# Autodesk Inventor assembly: Y Axis
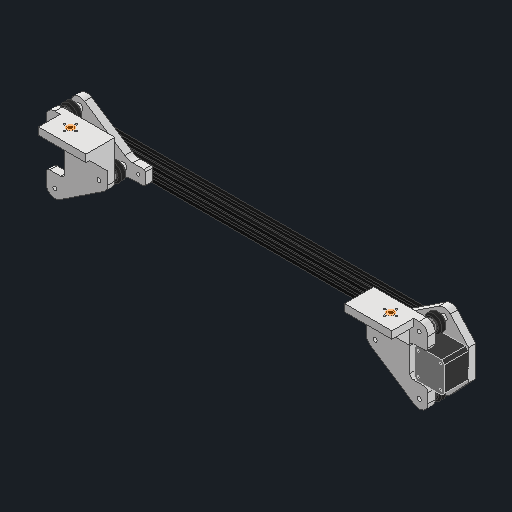
[picture p0: Inventor's stored thumbnail of the model, 512x512]
Saved by Autodesk Inventor 2025.1 (Build 291241000, 241)
## iProperties
Created: 2025-02-05
Part Number: Y Axis
Document SubType Name: Assembly
Designer: jerem
Author: jerem
## Documents named in this file (10)
- C:\Users\jerem\Documents\GitHub\Perovskite-Automated-Synthesis-System\CAD\Gantry\Y Axis.iam
- C:\Users\jerem\Documents\GitHub\Perovskite-Automated-Synthesis-System\CAD\Non 3D Printed Parts\Extrusion\V Extrustion 20x500mm.ipt
- C:\Users\jerem\Documents\GitHub\Perovskite-Automated-Synthesis-System\CAD\Gantry\y axis motor holder.ipt
- C:\Users\jerem\Documents\GitHub\Perovskite-Automated-Synthesis-System\CAD\Gantry\y axis something back.ipt
- C:\Users\jerem\Documents\GitHub\Perovskite-Automated-Synthesis-System\CAD\Gantry\y axis something.ipt
- C:\Users\jerem\Documents\GitHub\Perovskite-Automated-Synthesis-System\CAD\Non 3D Printed Parts\Motors and Servos\NEMA17 Stepper Motor.ipt
- C:\Users\jerem\Documents\GitHub\Perovskite-Automated-Synthesis-System\CAD\Non 3D Printed Parts\Printer Wheel.ipt
- C:\Users\jerem\Documents\GitHub\Perovskite-Automated-Synthesis-System\CAD\Gantry\y axis something_MIR.ipt
- C:\Users\jerem\Documents\GitHub\Perovskite-Automated-Synthesis-System\CAD\Non 3D Printed Parts\Leadscrew.ipt
- C:\Users\jerem\Documents\GitHub\Perovskite-Automated-Synthesis-System\CAD\Gantry\Y Axis Spacer.ipt
## Components (26 placed, 9 different names)
1. V Extrustion 20x500mm:1 — Mate:14, Mate:24, Mate:25, Mate:26, Flush:1
2. y axis motor holder:1 — Mate:1, Mate:2, Mate:4, Mate:5, Mate:7, Mate:8, Mate:9, Mate:13, Mate:14, Mate:25, Mate:36, Mate:37, Mate:38, Mate:49, Mate:50, Flush:1
3. y axis something back:1 — Mate:21, Mate:22, Mate:24, Mate:26, Mate:39, Mate:40, Mate:41, Mate:58, Mate:59, Mate:60
4. y axis something:1 — Mate:4, Mate:5, Mate:30, Mate:31, Mate:32, Mate:33, Mate:34, Mate:35, Mate:46, Mate:47, Mate:48
5. NEMA17 Stepper Motor:1 — Mate:1, Mate:2, Mate:13
6. Printer Wheel:1 — Mate:7, Mate:54
7. Printer Wheel:2 — Mate:8, Mate:53
8. Printer Wheel:3 — Mate:9, Mate:45, Mate:51, Mate:52
9. y axis something_MIR:1 — Mate:16, Mate:17, Mate:18, Mate:21, Mate:22, Mate:27, Mate:28, Mate:29, Mate:42, Mate:43, Mate:44, Mate:55, Mate:56, Mate:57
10. Printer Wheel:4 — Mate:18, Mate:63, Mate:64
11. Printer Wheel:5 — Mate:17, Mate:62
12. Printer Wheel:6 — Mate:16, Mate:61
13. Leadscrew:1 — Mate:27, Mate:28, Mate:29
14. Leadscrew:2 — Mate:30, Mate:31, Mate:32
15. Y Axis Spacer:1 — Mate:37, Mate:49, Mate:54
16. Y Axis Spacer:2 — Mate:38, Mate:50, Mate:53
17. Y Axis Spacer:3 — Mate:36, Mate:45, Mate:51
18. Y Axis Spacer:4 — Mate:41, Mate:59, Mate:64
19. Y Axis Spacer:5 — Mate:43, Mate:55, Mate:62
20. Y Axis Spacer:6 — Mate:42, Mate:56, Mate:61
21. Y Axis Spacer:7 — Mate:40, Mate:58
22. Y Axis Spacer:8 — Mate:39, Mate:60
23. Y Axis Spacer:9 — Mate:44, Mate:57, Mate:63
24. Y Axis Spacer:10 — Mate:34, Mate:47
25. Y Axis Spacer:11 — Mate:35, Mate:46, Mate:52
26. Y Axis Spacer:12 — Mate:33, Mate:48
## Relationships (56: Mate 55, Flush 1)
- Mate:1: y axis motor holder:1 ↔ NEMA17 Stepper Motor:1
- Mate:2: y axis motor holder:1 ↔ NEMA17 Stepper Motor:1
- Mate:4: y axis motor holder:1 ↔ y axis something:1
- Mate:5: y axis motor holder:1 ↔ y axis something:1
- Mate:7: y axis motor holder:1 ↔ Printer Wheel:1
- Mate:8: y axis motor holder:1 ↔ Printer Wheel:2
- Mate:9: y axis motor holder:1 ↔ Printer Wheel:3
- Mate:13: y axis motor holder:1 ↔ NEMA17 Stepper Motor:1
- Mate:14: V Extrustion 20x500mm:1 ↔ y axis motor holder:1
- Mate:16: y axis something_MIR:1 ↔ Printer Wheel:6
- Mate:17: y axis something_MIR:1 ↔ Printer Wheel:5
- Mate:18: y axis something_MIR:1 ↔ Printer Wheel:4
- Mate:21: y axis something back:1 ↔ y axis something_MIR:1
- Mate:22: y axis something back:1 ↔ y axis something_MIR:1
- Mate:24: V Extrustion 20x500mm:1 ↔ y axis something back:1
- Mate:25: V Extrustion 20x500mm:1 ↔ y axis motor holder:1
- Mate:26: V Extrustion 20x500mm:1 ↔ y axis something back:1
- Mate:27: y axis something_MIR:1 ↔ Leadscrew:1
- Mate:28: y axis something_MIR:1 ↔ Leadscrew:1
- Mate:29: y axis something_MIR:1 ↔ Leadscrew:1
- Mate:30: y axis something:1 ↔ Leadscrew:2
- Mate:31: y axis something:1 ↔ Leadscrew:2
- Mate:32: y axis something:1 ↔ Leadscrew:2
- Mate:33: y axis something:1 ↔ Y Axis Spacer:12
- Mate:34: y axis something:1 ↔ Y Axis Spacer:10
- Mate:35: y axis something:1 ↔ Y Axis Spacer:11
- Mate:36: y axis motor holder:1 ↔ Y Axis Spacer:3
- Mate:37: y axis motor holder:1 ↔ Y Axis Spacer:1
- Mate:38: y axis motor holder:1 ↔ Y Axis Spacer:2
- Mate:39: y axis something back:1 ↔ Y Axis Spacer:8
- Mate:40: y axis something back:1 ↔ Y Axis Spacer:7
- Mate:41: y axis something back:1 ↔ Y Axis Spacer:4
- Mate:42: y axis something_MIR:1 ↔ Y Axis Spacer:6
- Mate:43: y axis something_MIR:1 ↔ Y Axis Spacer:5
- Mate:44: y axis something_MIR:1 ↔ Y Axis Spacer:9
- Mate:45: Printer Wheel:3 ↔ Y Axis Spacer:3
- Mate:46: y axis something:1 ↔ Y Axis Spacer:11
- Mate:47: y axis something:1 ↔ Y Axis Spacer:10
- Mate:48: y axis something:1 ↔ Y Axis Spacer:12
- Mate:49: y axis motor holder:1 ↔ Y Axis Spacer:1
- Mate:50: y axis motor holder:1 ↔ Y Axis Spacer:2
- Mate:51: Printer Wheel:3 ↔ Y Axis Spacer:3
- Mate:52: Printer Wheel:3 ↔ Y Axis Spacer:11
- Mate:53: Printer Wheel:2 ↔ Y Axis Spacer:2
- Mate:54: Printer Wheel:1 ↔ Y Axis Spacer:1
- Mate:55: y axis something_MIR:1 ↔ Y Axis Spacer:5
- Mate:56: y axis something_MIR:1 ↔ Y Axis Spacer:6
- Mate:57: y axis something_MIR:1 ↔ Y Axis Spacer:9
- Mate:58: y axis something back:1 ↔ Y Axis Spacer:7
- Mate:59: y axis something back:1 ↔ Y Axis Spacer:4
- Mate:60: y axis something back:1 ↔ Y Axis Spacer:8
- Mate:61: Printer Wheel:6 ↔ Y Axis Spacer:6
- Mate:62: Printer Wheel:5 ↔ Y Axis Spacer:5
- Mate:63: Printer Wheel:4 ↔ Y Axis Spacer:9
- Mate:64: Printer Wheel:4 ↔ Y Axis Spacer:4
- Flush:1: V Extrustion 20x500mm:1 ↔ y axis motor holder:1
